# Autodesk Inventor assembly: Wall Cabinet 2 Door with open shelf
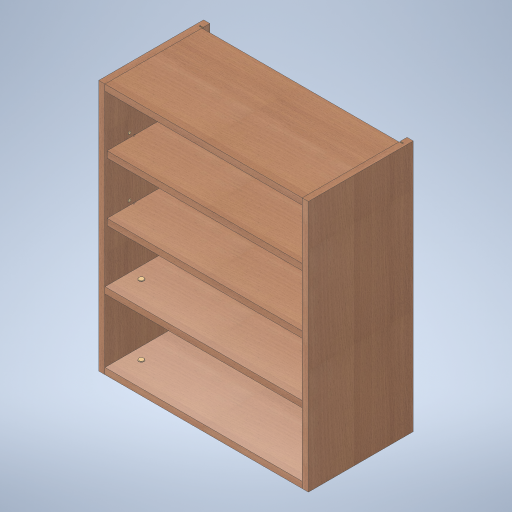
[picture p0: Inventor's stored thumbnail of the model, 512x512]
Saved by Autodesk Inventor 2024 (Build 280153000, 153)
## iProperties
RuleStatus: InUse
Created: 2017-01-26
Part Number: Wall Cabinet 2 Door with open shelf
Document SubType Name: Assembly
Designer: SvetlanaB
Author: SvetlanaB
## Documents named in this file (14)
- C:\W4INV 2024 Design\iBOX LIBRARY\Kitchen\Wall Cabinets\Cabinet with open shelf\Cabinet with open shelf.iam
- C:\W4INV 2024 Design\iBOX LIBRARY\Kitchen\Wall Cabinets\Cabinet with open shelf\Back panel.ipt
- C:\W4INV 2024 Design\iBOX LIBRARY\Kitchen\Wall Cabinets\Cabinet with open shelf\Shelf.ipt
- C:\W4INV 2024 Design\iBOX LIBRARY\Kitchen\Wall Cabinets\Cabinet with open shelf\Bottom shelf.ipt
- C:\W4INV 2024 Design\iBOX LIBRARY\Kitchen\Wall Cabinets\Cabinet with open shelf\Left panel.ipt
- C:\W4INV 2024 Design\iBOX LIBRARY\Kitchen\Wall Cabinets\Cabinet with open shelf\Bottom panel.ipt
- C:\W4INV 2024 Design\iBOX LIBRARY\Kitchen\Wall Cabinets\Cabinet with open shelf\Top panel.ipt
- C:\W4INV 2024 Design\iBOX LIBRARY\Kitchen\Wall Cabinets\Cabinet with open shelf\Right panel.ipt
- C:\W4INV 2024 Design\iBOX LIBRARY\Kitchen\Wall Cabinets\Cabinet with open shelf\2 Door open shelf cab skeleton.ipt
- C:\W4INV 2024 Design\_LIBRARY\Fixed joints\Minifix joint\MINIFIX D15 v2\Minifix D15 & Dowel L34 & Cap D15 PB T18 LH.ipt
- C:\W4INV 2024 Design\_LIBRARY\Holders\Shelf holder D5\Shelf support D5 L16 with hole covers.ipt
- C:\W4INV 2024 Design\_LIBRARY\Fixed joints\Minifix joint\MINIFIX D15 v2\Minifix D15 & Dowel L34 & Cap D15 PB T18 RH.ipt
- C:\W4INV 2023 Design\LIBRARY\Fixed joints\Minifix joint\MINIFIX D15 v2.ipt
- C:\W4INV 2023 Design\LIBRARY\Holders\Shelf holder D5.ipt
## Components (29 placed, 11 different names)
1. @Skeleton
2. Back panel:1
3. Bottom shelf:1 — Pillar Board Side Plane :9, Pillar Board Side Plane :10, Pillar Board Side Plane :11, Pillar Board Side Plane :12
4. Left panel:1 — Flush:1, Flush:2, Nestled Board Plane:1, Nestled Board Plane:2, Nestled Board Plane:3, Nestled Board Plane:4, Side Board Plane:1, Side Board Plane:2, Nestled Board Plane:9, Nestled Board Plane:11
5. Bottom panel:1 — Pillar Board Side Plane :3, Pillar Board Side Plane :4, Pillar Board Side Plane :7, Pillar Board Side Plane :8
6. Top panel:1 — Pillar Board Side Plane :1, Pillar Board Side Plane :2, Pillar Board Side Plane :5, Pillar Board Side Plane :6
7. Right panel:1 — Nestled Board Plane:5, Nestled Board Plane:6, Nestled Board Plane:7, Nestled Board Plane:8, Side Board Plane:3, Side Board Plane:4, Nestled Board Plane:10, Nestled Board Plane:12
8. Minifix D15 & Dowel L34 & Cap D15 PB T18 RH:1 — Axis Plane:1, Nestled Board Plane:1, Pillar Board Side Plane :1
9. Minifix D15 & Dowel L34 & Cap D15 PB T18 LH:2 — Axis Plane:2, Nestled Board Plane:2, Pillar Board Side Plane :2
10. Minifix D15 & Dowel L34 & Cap D15 PB T18 LH:3 — Axis Plane:3, Nestled Board Plane:3, Pillar Board Side Plane :3
11. Minifix D15 & Dowel L34 & Cap D15 PB T18 RH:4 — Axis Plane:4, Nestled Board Plane:4, Pillar Board Side Plane :4
12. Minifix D15 & Dowel L34 & Cap D15 PB T18 LH:5 — Axis Plane:5, Nestled Board Plane:5, Pillar Board Side Plane :5
13. Minifix D15 & Dowel L34 & Cap D15 PB T18 RH:6 — Axis Plane:6, Nestled Board Plane:6, Pillar Board Side Plane :6
14. Minifix D15 & Dowel L34 & Cap D15 PB T18 LH:7 — Axis Plane:7, Nestled Board Plane:7, Pillar Board Side Plane :7
15. Minifix D15 & Dowel L34 & Cap D15 PB T18 RH:8 — Axis Plane:8, Nestled Board Plane:8, Pillar Board Side Plane :8
16. Minifix D15 & Dowel L34 & Cap D15 PB T18 LH:10 — Axis Plane:13, Nestled Board Plane:9, Pillar Board Side Plane :9
17. Minifix D15 & Dowel L34 & Cap D15 PB T18 RH:11 — Axis Plane:14, Nestled Board Plane:10, Pillar Board Side Plane :10
18. Minifix D15 & Dowel L34 & Cap D15 PB T18 RH:12 — Axis Plane:15, Nestled Board Plane:11, Pillar Board Side Plane :11
19. Minifix D15 & Dowel L34 & Cap D15 PB T18 LH:13 — Axis Plane:16, Nestled Board Plane:12, Pillar Board Side Plane :12
20. Shelf:1 — Shelf Pottom Plane:1, Shelf Pottom Plane:2, Shelf Pottom Plane:3, Shelf Pottom Plane:4
21. Shelf support D5 L16 with hole covers:13 — Axis Plane:9, Side Board Plane:1, Shelf Pottom Plane:1
22. Shelf support D5 L16 with hole covers:14 — Axis Plane:10, Side Board Plane:2, Shelf Pottom Plane:2
23. Shelf support D5 L16 with hole covers:15 — Axis Plane:11, Side Board Plane:3, Shelf Pottom Plane:3
24. Shelf support D5 L16 with hole covers:16 — Axis Plane:12, Side Board Plane:4, Shelf Pottom Plane:4
25. Shelf:2
26. Shelf support D5 L16 with hole covers:17
27. Shelf support D5 L16 with hole covers:18
28. Shelf support D5 L16 with hole covers:19
29. Shelf support D5 L16 with hole covers:20
## Component patterns: (2 elements, first: Shelf:1 + Shelf support D5 L16 with hole covers:13 + Shelf support D5 L16 with hole covers:14 + Shelf support D5 L16 with hole covers:15 + Shelf support D5 L16 with hole covers:16)
## Relationships (50: Mate 36, Flush 14)
- Flush:1 (-70 mm): Left panel:1
- Flush:2 (-70 mm): Left panel:1
- Axis Plane:1 [Mate]: Minifix D15 & Dowel L34 & Cap D15 PB T18 RH:1
- Nestled Board Plane:1 [Mate]: Left panel:1 ↔ Minifix D15 & Dowel L34 & Cap D15 PB T18 RH:1
- Pillar Board Side Plane :1 [Flush] (18 mm): Top panel:1 ↔ Minifix D15 & Dowel L34 & Cap D15 PB T18 RH:1
- Axis Plane:2 [Mate]: Minifix D15 & Dowel L34 & Cap D15 PB T18 LH:2
- Nestled Board Plane:2 [Mate]: Left panel:1 ↔ Minifix D15 & Dowel L34 & Cap D15 PB T18 LH:2
- Pillar Board Side Plane :2 [Flush] (18 mm): Top panel:1 ↔ Minifix D15 & Dowel L34 & Cap D15 PB T18 LH:2
- Axis Plane:3 [Mate]: Minifix D15 & Dowel L34 & Cap D15 PB T18 LH:3
- Nestled Board Plane:3 [Mate]: Left panel:1 ↔ Minifix D15 & Dowel L34 & Cap D15 PB T18 LH:3
- Pillar Board Side Plane :3 [Flush] (18 mm): Bottom panel:1 ↔ Minifix D15 & Dowel L34 & Cap D15 PB T18 LH:3
- Axis Plane:4 [Mate]: Minifix D15 & Dowel L34 & Cap D15 PB T18 RH:4
- Nestled Board Plane:4 [Mate]: Left panel:1 ↔ Minifix D15 & Dowel L34 & Cap D15 PB T18 RH:4
- Pillar Board Side Plane :4 [Flush] (18 mm): Bottom panel:1 ↔ Minifix D15 & Dowel L34 & Cap D15 PB T18 RH:4
- Axis Plane:5 [Mate]: Minifix D15 & Dowel L34 & Cap D15 PB T18 LH:5
- Nestled Board Plane:5 [Mate]: Right panel:1 ↔ Minifix D15 & Dowel L34 & Cap D15 PB T18 LH:5
- Pillar Board Side Plane :5 [Flush] (18 mm): Top panel:1 ↔ Minifix D15 & Dowel L34 & Cap D15 PB T18 LH:5
- Axis Plane:6 [Mate]: Minifix D15 & Dowel L34 & Cap D15 PB T18 RH:6
- Nestled Board Plane:6 [Mate]: Right panel:1 ↔ Minifix D15 & Dowel L34 & Cap D15 PB T18 RH:6
- Pillar Board Side Plane :6 [Flush] (18 mm): Top panel:1 ↔ Minifix D15 & Dowel L34 & Cap D15 PB T18 RH:6
- Axis Plane:7 [Mate]: Minifix D15 & Dowel L34 & Cap D15 PB T18 LH:7
- Nestled Board Plane:7 [Mate]: Right panel:1 ↔ Minifix D15 & Dowel L34 & Cap D15 PB T18 LH:7
- Pillar Board Side Plane :7 [Flush] (18 mm): Bottom panel:1 ↔ Minifix D15 & Dowel L34 & Cap D15 PB T18 LH:7
- Axis Plane:8 [Mate]: Minifix D15 & Dowel L34 & Cap D15 PB T18 RH:8
- Nestled Board Plane:8 [Mate]: Right panel:1 ↔ Minifix D15 & Dowel L34 & Cap D15 PB T18 RH:8
- Pillar Board Side Plane :8 [Flush] (18 mm): Bottom panel:1 ↔ Minifix D15 & Dowel L34 & Cap D15 PB T18 RH:8
- Axis Plane:9 [Mate]: Shelf support D5 L16 with hole covers:13
- Side Board Plane:1 [Mate]: Left panel:1 ↔ Shelf support D5 L16 with hole covers:13
- Shelf Pottom Plane:1 [Mate] (2.5 mm): Shelf:1 ↔ Shelf support D5 L16 with hole covers:13
- Axis Plane:10 [Mate]: Shelf support D5 L16 with hole covers:14
- Side Board Plane:2 [Mate]: Left panel:1 ↔ Shelf support D5 L16 with hole covers:14
- Shelf Pottom Plane:2 [Mate] (2.5 mm): Shelf:1 ↔ Shelf support D5 L16 with hole covers:14
- Axis Plane:11 [Mate]: Shelf support D5 L16 with hole covers:15
- Side Board Plane:3 [Mate]: Right panel:1 ↔ Shelf support D5 L16 with hole covers:15
- Shelf Pottom Plane:3 [Mate] (2.5 mm): Shelf:1 ↔ Shelf support D5 L16 with hole covers:15
- Axis Plane:12 [Mate]: Shelf support D5 L16 with hole covers:16
- Side Board Plane:4 [Mate]: Right panel:1 ↔ Shelf support D5 L16 with hole covers:16
- Shelf Pottom Plane:4 [Mate] (2.5 mm): Shelf:1 ↔ Shelf support D5 L16 with hole covers:16
- Axis Plane:13 [Mate]: Minifix D15 & Dowel L34 & Cap D15 PB T18 LH:10
- Nestled Board Plane:9 [Mate]: Left panel:1 ↔ Minifix D15 & Dowel L34 & Cap D15 PB T18 LH:10
- Pillar Board Side Plane :9 [Flush] (18 mm): Bottom shelf:1 ↔ Minifix D15 & Dowel L34 & Cap D15 PB T18 LH:10
- Axis Plane:14 [Mate]: Minifix D15 & Dowel L34 & Cap D15 PB T18 RH:11
- Nestled Board Plane:10 [Mate]: Right panel:1 ↔ Minifix D15 & Dowel L34 & Cap D15 PB T18 RH:11
- Pillar Board Side Plane :10 [Flush] (18 mm): Bottom shelf:1 ↔ Minifix D15 & Dowel L34 & Cap D15 PB T18 RH:11
- Axis Plane:15 [Mate]: Minifix D15 & Dowel L34 & Cap D15 PB T18 RH:12
- Nestled Board Plane:11 [Mate]: Left panel:1 ↔ Minifix D15 & Dowel L34 & Cap D15 PB T18 RH:12
- Pillar Board Side Plane :11 [Flush] (18 mm): Bottom shelf:1 ↔ Minifix D15 & Dowel L34 & Cap D15 PB T18 RH:12
- Axis Plane:16 [Mate]: Minifix D15 & Dowel L34 & Cap D15 PB T18 LH:13
- Nestled Board Plane:12 [Mate]: Right panel:1 ↔ Minifix D15 & Dowel L34 & Cap D15 PB T18 LH:13
- Pillar Board Side Plane :12 [Flush] (18 mm): Bottom shelf:1 ↔ Minifix D15 & Dowel L34 & Cap D15 PB T18 LH:13
## Named parameters: Shelf_quantity = 2, Panel_thickness = 18 mm, Open_Shelf_Space = 200 mm, Distance_between_shelfs = 149.33333 mm
